# Autodesk Inventor assembly: Motor with Cover
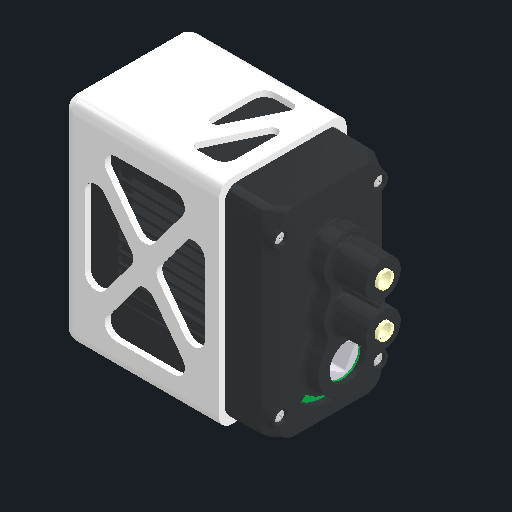
[picture p0: Inventor's stored thumbnail of the model, 512x512]
Saved by Autodesk Inventor 2025 (Build 290162000, 162)
## iProperties
Created: 2025-01-27
Part Number: Motor with Cover
Document SubType Name: Assembly
Designer: Averey Ku
Author: Averey Ku
## Documents named in this file (3)
- D:\VEX\High Stakes\CAD\V5\Chassis\Drivebay Right\Motor with Cover.iam
- D:\VEX\High Stakes\CAD\V5\Chassis\Drivebay Right\V5 Motor.ipt
- D:\VEX\High Stakes\CAD\V5\Chassis\Drivebay Right\Motor Cover.ipt
## Components (2 placed, 2 different names)
1. V5 Motor:1 — Mate:2, Mate:1
2. Motor Cover:1 — Mate:2, Mate:1
## Relationships (2: Mate 2)
- Mate:2: V5 Motor:1 ↔ Motor Cover:1
- Mate:1: V5 Motor:1 ↔ Motor Cover:1
